# Autodesk Inventor assembly: layer 2 + horn
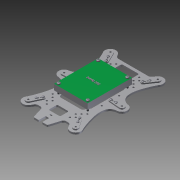
[picture p0: Inventor's stored thumbnail of the model, 180x180]
Saved by Autodesk Inventor 2012 (Build 160160000, 160)
## iProperties
Created: 2013-12-07
Part Number: layer 2 + horn
Document SubType Name: Assembly
Designer: Irwan Haryanto
Author: Irwan Haryanto
## Documents named in this file (9)
- D:\Revenant\robot baru 2014\layer 2 + horn.iam
- D:\Revenant\robot baru 2014\layer 2.ipt
- D:\Revenant\robot baru 2014\Horn.ipt
- D:\Revenant\robot baru 2014\layer 2 + horn\Design Accelerator\Bolted Connection1.iam
- D:\Revenant\robot baru 2014\ssc board.ipt
- D:\Revenant\robot baru 2014\layer 2 + horn\Design Accelerator\Bolted Connection6.iam
- D:\Revenant\robot baru 2014\layer 2 + horn\Design Accelerator\Bolted Connection7.iam
- D:\Revenant\robot baru 2014\layer 2 + horn\Design Accelerator\Bolted Connection8.iam
- D:\Revenant\robot baru 2014\layer 2 + horn\Design Accelerator\Bolted Connection9.iam
## Components (13 placed, 4 different names)
1. layer 2:1 — Insert:1, Insert:2, Insert:3, Insert:4, Insert:5, Insert:6, Insert:7, Insert:8, Insert:9, Insert:10, Insert:11, Insert:12, Insert:13, Mate:2, Insert:14, Insert:15, Mate:4, Mate:6, Mate:8, Mate:10
2. Horn:1 — Insert:1, Insert:2, Insert:3, Mate:1
3. Horn:2 — Insert:4, Insert:5
4. Horn:3 — Insert:6, Insert:7
5. Horn:4 — Insert:8, Insert:9
6. Horn:5 — Insert:10, Insert:11
7. Horn:6 — Insert:12, Insert:13
8. Bolted Connection:1 [sub-assembly] — Mate:1, Mate:2
9. ssc board:1 — Insert:14, Insert:15, Mate:3, Mate:5, Mate:7, Mate:9
10. Bolted Connection:2 [sub-assembly] — Mate:3, Mate:4
11. Bolted Connection:3 [sub-assembly] — Mate:5, Mate:6
12. Bolted Connection:4 [sub-assembly] — Mate:7, Mate:8
13. Bolted Connection:5 [sub-assembly] — Mate:9, Mate:10
## Relationships (25: Insert 15, Mate 10)
- Insert:1: layer 2:1 ↔ Horn:1
- Insert:2: layer 2:1 ↔ Horn:1
- Insert:3: layer 2:1 ↔ Horn:1
- Insert:4: layer 2:1 ↔ Horn:2
- Insert:5: layer 2:1 ↔ Horn:2
- Insert:6: layer 2:1 ↔ Horn:3
- Insert:7: layer 2:1 ↔ Horn:3
- Insert:8: layer 2:1 ↔ Horn:4
- Insert:9: layer 2:1 ↔ Horn:4
- Insert:10: layer 2:1 ↔ Horn:5
- Insert:11: layer 2:1 ↔ Horn:5
- Insert:12: layer 2:1 ↔ Horn:6
- Insert:13: layer 2:1 ↔ Horn:6
- Mate:1: Horn:1 ↔ Bolted Connection:1
- Mate:2: layer 2:1 ↔ Bolted Connection:1
- Insert:14 (5 mm): layer 2:1 ↔ ssc board:1
- Insert:15 (5 mm): layer 2:1 ↔ ssc board:1
- Mate:3: ssc board:1 ↔ Bolted Connection:2
- Mate:4: layer 2:1 ↔ Bolted Connection:2
- Mate:5: ssc board:1 ↔ Bolted Connection:3
- Mate:6: layer 2:1 ↔ Bolted Connection:3
- Mate:7: ssc board:1 ↔ Bolted Connection:4
- Mate:8: layer 2:1 ↔ Bolted Connection:4
- Mate:9: ssc board:1 ↔ Bolted Connection:5
- Mate:10: layer 2:1 ↔ Bolted Connection:5
